# Autodesk Inventor assembly: robot
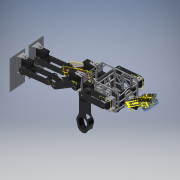
[picture p0: Inventor's stored thumbnail of the model, 180x180]
Saved by Autodesk Inventor 2018 (Build 220112000, 112)
## iProperties
Created: 2018-11-26
Part Number: robot
Document SubType Name: Assembly
Designer: bitbots
Author: bitbots
## Documents named in this file (8)
- C:\Users\jaspe\gits\bitbots_hardware\wolfgang\assembly\robot.iam
- C:\Users\jaspe\gits\bitbots_hardware\wolfgang\assembly\legs\left_leg.iam
- C:\Users\jaspe\gits\bitbots_hardware\wolfgang\assembly\body\body_assembly.iam
- C:\Users\jaspe\gits\bitbots_hardware\wolfgang\assembly\legs\left_leg_MIR.iam
- C:\Users\jaspe\gits\bitbots_hardware\wolfgang\assembly\arms\left_arm.iam
- C:\Users\jaspe\gitss\bitbots_hardware\wolfgang\assembly\arms\right_arm.iam
- C:\Users\jaspe\gits\bitbots_hardware\wolfgang\assembly\head\head.iam
- head.iam
## Components (6 placed, 6 different names)
1. left_leg:1 [sub-assembly] — Mate:4, Mate:5, Mate:6
2. body_assembly:1 [sub-assembly] — Mate:4, Mate:5, Mate:6, Mate:7, Mate:8, Mate:9, Mate:10, Mate:11, Mate:12, Mate:13, Mate:14, Mate:15, Mate:16, Mate:17, Mate:18, Mate:19
3. left_leg_MIR:1 [sub-assembly] — Mate:7, Mate:8, Mate:9
4. left_arm:1 [sub-assembly] — Mate:11, Mate:14, Mate:15
5. right_arm:1 [sub-assembly] — Mate:10, Mate:12, Mate:13
6. head:1 [sub-assembly] — Mate:16, Mate:17, Mate:18, Mate:19
## Relationships (16: Mate 16)
- Mate:4: left_leg:1 ↔ body_assembly:1
- Mate:5: left_leg:1 ↔ body_assembly:1
- Mate:6: left_leg:1 ↔ body_assembly:1
- Mate:7: body_assembly:1 ↔ left_leg_MIR:1
- Mate:8: body_assembly:1 ↔ left_leg_MIR:1
- Mate:9: body_assembly:1 ↔ left_leg_MIR:1
- Mate:10: body_assembly:1 ↔ right_arm:1
- Mate:11: body_assembly:1 ↔ left_arm:1
- Mate:12: body_assembly:1 ↔ right_arm:1
- Mate:13: body_assembly:1 ↔ right_arm:1
- Mate:14: body_assembly:1 ↔ left_arm:1
- Mate:15: body_assembly:1 ↔ left_arm:1
- Mate:16: body_assembly:1 ↔ head:1
- Mate:17: body_assembly:1 ↔ head:1
- Mate:18: body_assembly:1 ↔ head:1
- Mate:19: body_assembly:1 ↔ head:1
